# Autodesk Inventor assembly: C-SXR24-160
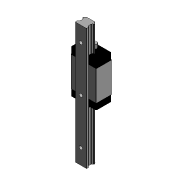
[picture p0: Inventor's stored thumbnail of the model, 180x180]
Saved by Autodesk Inventor 2020 (Build 240168000, 168)
## iProperties
Part Number: C-SXR24-160
Catalog Web Link: www.cadenas.de
Description: C-SXR, C-SX2R, C-SXRL, C-SX2RL-C-VALUE Linear Guides for Heavy Load
Vendor: MISUMI
Document SubType Name: Assembly
Designer: partserver
Manufacturer: MISUMI
Mass: 57.6648 g
Surface Area: 189.482 cm^2
Volume: 57.6648 cm^3
Density: 1 g/cm^3
Category: PARTsolutions
Company: MISUMI
PSOL_IDENT_0: {$CADENAS_DATA\23d-libs\misumi\metric\06_linear_guides\06_cn\c_sxr_asmtab.prj},215 {VTYP=3D},{STYP=A
PSOL_IDENT_1: SSTAB},{NB=C-SXR24-160},{LINA=C-SXR24-160},{NN=C-SXR, C-SX2R, C-SXRL, C-SX2RL},{DATE=20.05.2021 06:4
PSOL_IDENT_2: 3:21},{GEOMDATE=11.06.2020 08:16:51},{VERSION=},{LINEID=10},{WBVAR=NOB,LT,LS,ALT},{WBNUMERIC=LS}  {N
PSOL_IDENT_3: B=C-SXR24-160},{LINA=C-SXR24-160},{KT=DUMMY},{PN=C-SXR24-160},{TYPE=C-SX},{H=24},{NOB=},{LT=},{LS=16
PSOL_IDENT_4: 0},{LALG=[100,160,220,280,340,400,460,520,580,640,700,760,820,880,940,1000,1060,1120,1180,1240,1300,
PSOL_IDENT_5: 1360,1420,1480]},{LSALG=[100,160,220,280,340,400,460,520,580,640,700,760,820,880,940,1000,1060,1120,
PSOL_IDENT_6: 1180,1240,1300,1360,1420,1480]},{LALG0=[110:150/10],[170:210/10],[230:270/10],[290:330/10],[350:390/
PSOL_IDENT_7: 10],[410:450/10],[470:510/10],[530:570/10],[590:630/10],[650:690/10],[710:750/10],[770:810/10],[830:
PSOL_IDENT_8: 870/10],[890:930/10],[950:990/10],[1010:1050/10],[1070:1110/10],[1130:1170/10],[1190:1230/10],[1250:
PSOL_IDENT_9: 1290/10],[1310:1350/10],[1370:1410/10],[1430:1470/10]},{LMIN=110},{LMAX=1470},{W=34},{L1=55.9},{B=26
PSOL_IDENT_10: },{C=26},{S=4.000},{LL=5.000},{SLL=M4x5},{L2=39.5},{K=20.8},{T=6.20},{CBB=0.5},{E=7},{T1=5.5},{H1=13
PSOL_IDENT_11: .0},{W1=15},{W2=9.5},{CAA=0.5},{DD1=4.5},{DD2=7.5},{HH=6.0},{DDH=4.5x7.5x6},{F=60},{G=20},{LW1=7.217
PSOL_IDENT_12: },{LW2=11.000},{LH1=8.221},{LH2=4.659},{LH3=3.221},{LH4=4.700},{LC1=0.300},{LC2=2.000},{LC3=0.500},{
PSOL_IDENT_13: LR1=1.431},{LR2=0.300},{LR3=0.300},{LR4=0.300},{M=3},{ALT=},{ALTALG= '','Not applicable' },{NL=0},{P
PSOL_IDENT_14: PATH=c_sxr/c_sxr_asmtpl.prj}
NB: C-SXR24-160
NN: C-SXR, C-SX2R, C-SXRL, C-SX2RL
NT: C-VALUE Linear Guides for Heavy Load
NBSYN: $PN.
LINA: C-SXR24-160
CATALOG: Misumi
PN: C-SXR24-160
H: 24
NOB: 1
LT: Selectable
LS: 160
W: 34
L1: 55.9
B: 26
C: 26
SLL: M4x5
L2: 39.5
K: 20.8
T: 6.2
CBB: 0.5
E: 7
T1: 5.5
H1: 13
W1: 15
W2: 9.5
CAA: 0.5
DDH: 4.5x7.5x6
F: 60
G: 20
ALT: Not applicable
SUPPLIER: MISUMI
ARTICLENO: C-SXR24-160
BOMINFO: C-SXR24-160
CREATOR: CADENAS GmbH
Title: C-SXR24-160
Author: Cadenas PARTsolutions
Comments: C-VALUE Linear Guides for Heavy Load
## Documents named in this file (3)
- C:\Users\lvglv\Documents\GitHub\Vibration_Generator\Parts\MISUMI\C-SXR24-160_Autodesk_Inventor_2020_20210817\AIS2020\C-SXR24-160.iam
- C:\Users\lvglv\Documents\GitHub\Vibration_Generator\Parts\MISUMI\C-SXR24-160_Autodesk_Inventor_2020_20210817\AIS2020\C-SXR24-160_r.ipt
- C:\Users\lvglv\Documents\GitHub\Vibration_Generator\Parts\MISUMI\C-SXR24-160_Autodesk_Inventor_2020_20210817\AIS2020\C-SXR24-R_b.ipt
## Components (2 placed, 2 different names)
1. C-SXR24-160_r:1 — to_block_1_Z@1 <-> to_rail_Z@2, to_block_1_YZ@1 <-> to_rail_YZ@2
2. C-SXR24-R_b:1 — to_block_1_Z@1 <-> to_rail_Z@2, to_block_1_YZ@1 <-> to_rail_YZ@2
## Relationships (2: Mate 1, Angle 1)
- to_block_1_Z@1 <-> to_rail_Z@2 [Mate]: C-SXR24-160_r:1 ↔ C-SXR24-R_b:1
- to_block_1_YZ@1 <-> to_rail_YZ@2 [Angle] (180 deg): C-SXR24-160_r:1 ↔ C-SXR24-R_b:1
